# Autodesk Inventor assembly: tiangsprayer
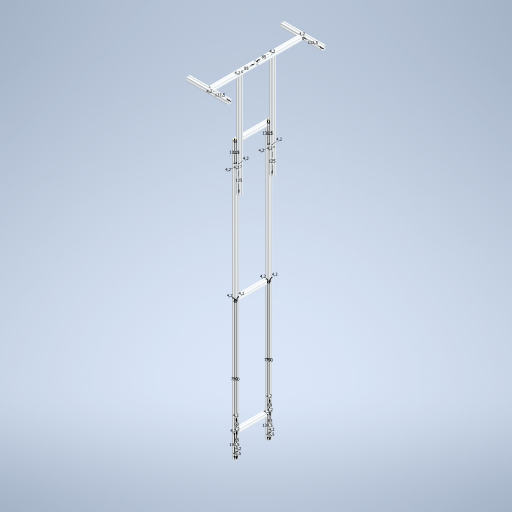
[picture p0: Inventor's stored thumbnail of the model, 512x512]
Saved by Autodesk Inventor 2023 (Build 270158000, 158)
## iProperties
Created: 2023-10-16
Part Number: tiangsprayer
Document SubType Name: Assembly
Designer: sigit
Author: sigit
## Documents named in this file (6)
- D:\Kuliah\SEMESTER 7\Robot Semprot\Design\REVISI2\Assembly\tiangsprayer.iam
- D:\Kuliah\SEMESTER 7\Robot Semprot\Design\REVISI2\Part\2020 560.ipt
- D:\Kuliah\SEMESTER 7\Robot Semprot\Design\2nd ROBOT\Part\2020 1500.ipt
- D:\Kuliah\SEMESTER 7\Robot Semprot\Design\2nd ROBOT\Part\2020 160.ipt
- D:\Kuliah\SEMESTER 7\Robot Semprot\Design\2nd ROBOT\Part\2020 240.ipt
- D:\Kuliah\SEMESTER 7\Robot Semprot\Design\2nd ROBOT\Part\2020 225.ipt
## Components (11 placed, 5 different names)
1. 2020 160:3 — Rotational:3
2. 2020 240:1 — Rotational:4, Rotational:5
3. 2020 225:1 — Rotational:5
4. 2020 240:2 — Rotational:7
5. 2020 225:2
6. 2020 1500:1 — Rotational:1, Rotational:2, Rotational:3
7. 2020 560:1 — Rotational:1, Rotational:7
8. 2020 1500:2
9. 2020 560:2 — Rotational:4
10. 2020 160:1 — Rotational:2
11. 2020 160:2
## Component patterns: (2 elements, first: 2020 1500:1 + 2020 560:1), (2 elements, first: 2020 160:1)
## Relationships (7: RevoluteJoint 7)
- Rotational:1 [RevoluteJoint] (12.2 mm): 2020 1500:1 ↔ 2020 560:1
- Rotational:2 [RevoluteJoint] (6.1 mm): 2020 1500:1 ↔ 2020 160:1
- Rotational:3 [RevoluteJoint] (6.1 mm): 2020 160:3 ↔ 2020 1500:1
- Rotational:4 [RevoluteJoint] (-6.1 mm): 2020 240:1 ↔ 2020 560:2
- Rotational:5 [RevoluteJoint] (-6.1 mm): 2020 240:1 ↔ 2020 225:1
- [RevoluteJoint] (-6.1 mm): 2020 240:2 ↔ 2020 225:2
- Rotational:7 [RevoluteJoint] (-12.2 mm): 2020 240:2 ↔ 2020 560:1
## Named parameters: d18_d16 = -6.1 mm, d19_d17 = 0 deg
